# Autodesk Inventor assembly: TS_V1_Fallmagazin_gesamt
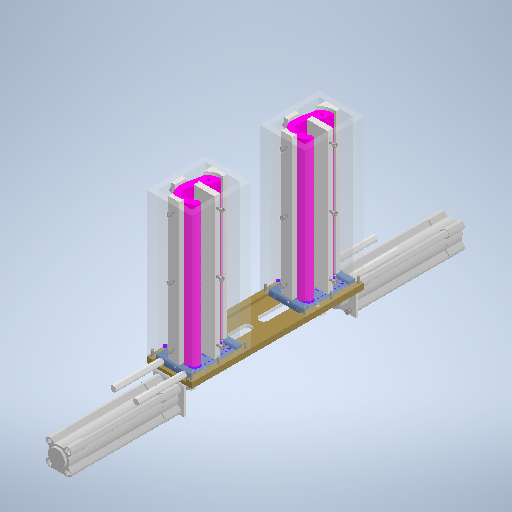
[picture p0: Inventor's stored thumbnail of the model, 512x512]
Saved by Autodesk Inventor 2025.2 (Build 292293000, 293)
## iProperties
Created: 2025-06-10
Part Number: TS_V1_Fallmagazin_gesamt
Document SubType Name: Assembly
Designer: tino
Author: tino
## Documents named in this file (16)
- C:\Users\tino\Documents_VM\Konstruieren_CAD\Useless Box\Eigene Bauteile\TS_V1_Fallmagazin_gesamt.iam
- C:\Users\tino\Documents_VM\Konstruieren_CAD\Useless Box\Eigene Bauteile\TS_V1_Fallmagazin_Boden_int.ipt
- C:\Users\tino\Documents_VM\Konstruieren_CAD\Useless Box\Eigene Bauteile\TS_V1_Fallmagazin_Wandung_int.ipt
- C:\Users\tino\Documents_VM\Konstruieren_CAD\Useless Box\Eigene Bauteile\TS_V1_Fallmagazin_Leitbleche_vorne_int.ipt
- C:\Users\tino\Documents_VM\Konstruieren_CAD\Useless Box\_Useless_Box\Finger.ipt
- C:\Users\tino\Documents_VM\Konstruieren_CAD\Useless Box\Eigene Bauteile\TS_V1_Fallmagazin_Schieber.iam
- C:\Users\tino\Documents_VM\Konstruieren_CAD\Useless Box\Kaufteile\Festo_100mm\1376426 DSBC-32-100-PPVA-N3---(0).iam
- C:\Users\tino\Documents_VM\Konstruieren_CAD\Useless Box\Kaufteile\Festo_100mm\1376426 DSBC-32-100-PPVA-N3---(0)_MIR.iam
- C:\Users\tino\Documents_VM\Konstruieren_CAD\Useless Box\Standart Bauteile\ISO 4762 - M4 x 12ISO.ipt
- C:\Users\tino\Documents_VM\Konstruieren_CAD\Useless Box\Standart Bauteile\ISO 4762 - M4 x 16ISO.ipt
- C:\Users\tino\Documents_VM\Konstruieren_CAD\Useless Box\Eigene Bauteile\TS_V1_Fallmagazin_Zylinderanbindung_int.ipt
- C:\Users\tino\Documents_VM\Konstruieren_CAD\Useless Box\Eigene Bauteile\TS_V1_Fallmagazin_Stopper_int.ipt
- C:\Users\tino\Documents_VM\Konstruieren_CAD\Useless Box\Eigene Bauteile\TS_V1_Fallmagazin_Zylinderhalter_int.ipt
- C:\Users\tino\Documents_VM\Konstruieren_CAD\Useless Box\Standart Bauteile\ISO 4762 - M5 x 8ISO.ipt
- C:\Users\tino\Documents_VM\Konstruieren_CAD\Useless Box\Standart Bauteile\ISO 4762 - M5 x 20ISO.ipt
- C:\Users\tino\Documents_VM\Konstruieren_CAD\Useless Box\Standart Bauteile\DIN EN ISO 2338 - 4 m6 x 10.ipt
## Components (169 placed, 15 different names)
1. TS_V1_Fallmagazin_Boden_int:1 — Passend:16, Passend:17, Fluchtend:5, Passend:21, Passend:23, Passend:25, Passend:26, Passend:30, Passend:31, Passend:43, Passend:44, Passend:45, Passend:46, Fluchtend:13, Passend:51, Fluchtend:15, Passend:59, Passend:60, Fluchtend:18, Passend:78, Passend:79, Passend:84, Passend:85, Passend:86, Passend:87
2. TS_V1_Fallmagazin_Wandung_int:2 — Passend:7, Passend:8, Fluchtend:4, Winkel:1, Winkel:2, Passend:16, Passend:17, Fluchtend:5, Passend:35, Passend:36, Passend:37, Passend:38, Passend:39, Passend:40, Passend:41, Passend:42, Winkel:3
3. TS_V1_Fallmagazin_Leitbleche_vorne_int:1 — Passend:7, Passend:8, Fluchtend:4, Tangential:2, Tangential:5, Fluchtend:12
4. TS_V1_Fallmagazin_Schieber:1 [sub-assembly] — Passend:21, Passend:25, Passend:26, Passend:52, Passend:53, Passend:61, Passend:62, Passend:63, Passend:64
5. TS_V1_Fallmagazin_Schieber:2 [sub-assembly] — Passend:23, Passend:30, Passend:31, Passend:56, Passend:57, Passend:65, Passend:66, Passend:67
6. 1376426 DSBC-32-100-PPVA-N3---(0):1 [sub-assembly] — Passend:54, Passend:59, Fluchtend:17, Fluchtend:18, Passend:68, Passend:69, Passend:70
7. 1376426 DSBC-32-100-PPVA-N3---(0)_MIR:1 [sub-assembly] — Passend:51, Fluchtend:15, Passend:58, Passend:60, Fluchtend:17, Passend:75, Passend:76, Passend:77
8. TS_V1_Fallmagazin_Wandung_int:3 — Passend:45, Passend:46, Fluchtend:13, Passend:47, Fluchtend:14, Passend:48
9. TS_V1_Fallmagazin_Leitbleche_vorne_int:2 — Passend:47, Fluchtend:14, Passend:48
10. TS_V1_Fallmagazin_Zylinderanbindung_int:1 — Passend:52, Passend:53, Passend:54
11. TS_V1_Fallmagazin_Zylinderanbindung_int:2 — Passend:56, Passend:57, Passend:58
12. TS_V1_Fallmagazin_Stopper_int:1 — Passend:61, Passend:62, Winkel:3
13. TS_V1_Fallmagazin_Stopper_int:2 — Passend:63, Passend:64
14. TS_V1_Fallmagazin_Stopper_int:3 — Passend:65, Fluchtend:16, Passend:67
15. TS_V1_Fallmagazin_Stopper_int:4 — Passend:66, Fluchtend:16
16. TS_V1_Fallmagazin_Zylinderhalter_int:1 — Passend:68, Passend:69, Passend:70, Passend:71, Passend:72, Passend:73, Passend:74
17. TS_V1_Fallmagazin_Zylinderhalter_int:2 — Passend:75, Passend:76, Passend:77, Passend:78, Passend:79, Passend:80, Passend:81, Passend:82, Passend:83
18. DIN EN ISO 2338 4 m6 x 10:1 — Passend:84, Passend:85
19. DIN EN ISO 2338 4 m6 x 10:2 — Passend:86, Passend:87
20. Finger:1 — Winkel:1, Tangential:2, Tangential:5, Winkel:2, Fluchtend:12
21. Finger:2
22. Finger:3
23. Finger:4
24. Finger:5
25. Finger:6
26. Finger:7
27. Finger:8
28. Finger:9
29. Finger:10
30. Finger:11
31. Finger:12
32. Finger:13
33. Finger:14
34. Finger:15
35. Finger:16
36. Finger:17
37. Finger:18
38. Finger:19
39. Finger:20
40. Finger:21
41. Finger:22
42. Finger:23
43. Finger:24
44. Finger:25
45. Finger:26
46. Finger:27
47. Finger:28
48. Finger:29
49. Finger:30
50. Finger:31
51. Finger:32
52. Finger:33
53. Finger:34
54. Finger:35
55. Finger:36
56. Finger:37
57. Finger:38
58. Finger:39
59. Finger:40
60. Finger:41
61. Finger:42
62. Finger:43
63. Finger:44
64. Finger:45
65. Finger:46
66. Finger:47
67. Finger:48
68. Finger:49
69. Finger:50
70. Finger:51
71. Finger:52
72. Finger:53
73. Finger:54
74. Finger:55
75. Finger:56
76. Finger:57
77. Finger:58
78. Finger:59
79. Finger:60
80. Finger:61
81. Finger:62
82. Finger:63
83. Finger:64
84. Finger:65
85. Finger:66
86. Finger:67
87. Finger:68
88. Finger:69
89. Finger:70
90. Finger:71
91. Finger:72
92. Finger:73
93. Finger:74
94. Finger:75
95. Finger:76
96. Finger:77
97. Finger:78
98. Finger:79
99. Finger:80
100. Finger:81
101. Finger:82
102. Finger:83
103. Finger:84
104. Finger:85
105. Finger:86
106. Finger:87
107. Finger:88
108. Finger:89
109. Finger:90
110. Finger:91
111. Finger:92
112. Finger:93
113. Finger:94
114. Finger:95
115. Finger:96
116. Finger:97
117. Finger:98
118. ISO 4762 M5 x 8:1 — Passend:71, Passend:72
119. ISO 4762 M5 x 8:2
120. ISO 4762 M5 x 8:3
121. ISO 4762 M5 x 8:4
122. ISO 4762 M5 x 20:1 — Passend:73, Passend:74
123. ISO 4762 M5 x 20:2
124. ISO 4762 M5 x 20:3
125. ISO 4762 M5 x 20:4
126. ISO 4762 M5 x 8:5 — Passend:80, Passend:81
127. ISO 4762 M5 x 8:6
128. ISO 4762 M5 x 8:7
129. ISO 4762 M5 x 8:8
130. ISO 4762 M5 x 20:5 — Passend:82, Passend:83
131. ISO 4762 M5 x 20:6
132. ISO 4762 M5 x 20:7
133. ISO 4762 M5 x 20:8
134. ISO 4762 M4 x 12:1 — Passend:35, Passend:36
135. ISO 4762 M4 x 12:2
136. ISO 4762 M4 x 12:3
137. ISO 4762 M4 x 12:4 — Passend:37, Passend:38
138. ISO 4762 M4 x 12:5
139. ISO 4762 M4 x 12:6
140. ISO 4762 M4 x 12:7 — Passend:39, Passend:40
141. ISO 4762 M4 x 12:8
142. ISO 4762 M4 x 12:9
143. ISO 4762 M4 x 12:10 — Passend:41, Passend:42
144. ISO 4762 M4 x 12:11
145. ISO 4762 M4 x 12:12
146. ISO 4762 M4 x 16:1 — Passend:43, Passend:44
147. ISO 4762 M4 x 16:2
148. ISO 4762 M4 x 16:3
149. ISO 4762 M4 x 16:4
150. ISO 4762 M4 x 16:5
151. ISO 4762 M4 x 16:6
152. ISO 4762 M4 x 12:13
153. ISO 4762 M4 x 12:14
154. ISO 4762 M4 x 12:15
155. ISO 4762 M4 x 12:16
156. ISO 4762 M4 x 12:17
157. ISO 4762 M4 x 12:18
158. ISO 4762 M4 x 12:19
159. ISO 4762 M4 x 12:20
160. ISO 4762 M4 x 12:21
161. ISO 4762 M4 x 12:22
162. ISO 4762 M4 x 12:23
163. ISO 4762 M4 x 12:24
164. ISO 4762 M4 x 16:7
165. ISO 4762 M4 x 16:8
166. ISO 4762 M4 x 16:9
167. ISO 4762 M4 x 16:10
168. ISO 4762 M4 x 16:11
169. ISO 4762 M4 x 16:12
## Component patterns: (2 elements), (98 elements, first: Finger:1), (4 elements, first: ISO 4762 M5 x 8:1), (4 elements, first: ISO 4762 M5 x 20:1), (4 elements, first: ISO 4762 M5 x 8:5), (4 elements, first: ISO 4762 M5 x 20:5), (3 elements, first: ISO 4762 M4 x 12:1), (3 elements, first: ISO 4762 M4 x 12:4), (3 elements, first: ISO 4762 M4 x 12:7), (3 elements, first: ISO 4762 M4 x 12:10), (6 elements, first: ISO 4762 M4 x 16:1), Komponentenanordnung 2:2 (3 elements), Komponentenanordnung 3:2 (3 elements), Komponentenanordnung 4:2 (3 elements), Komponentenanordnung 5:2 (3 elements), Komponentenanordnung 6:2 (6 elements)
## Relationships (74: Mate 60, Flush 9, Angle 3, Tangent 2)
- Passend:7 [Mate]: TS_V1_Fallmagazin_Wandung_int:2 ↔ TS_V1_Fallmagazin_Leitbleche_vorne_int:1
- Passend:8 [Mate]: TS_V1_Fallmagazin_Wandung_int:2 ↔ TS_V1_Fallmagazin_Leitbleche_vorne_int:1
- Fluchtend:4 [Flush]: TS_V1_Fallmagazin_Wandung_int:2 ↔ TS_V1_Fallmagazin_Leitbleche_vorne_int:1
- Winkel:1 [Angle] (0 deg): TS_V1_Fallmagazin_Wandung_int:2 ↔ Finger:1
- Tangential:2: TS_V1_Fallmagazin_Leitbleche_vorne_int:1 ↔ Finger:1
- Tangential:5: TS_V1_Fallmagazin_Leitbleche_vorne_int:1 ↔ Finger:1
- Winkel:2 [Angle] (0 deg): TS_V1_Fallmagazin_Wandung_int:2 ↔ Finger:1
- Passend:16 [Mate]: TS_V1_Fallmagazin_Boden_int:1 ↔ TS_V1_Fallmagazin_Wandung_int:2
- Passend:17 [Mate]: TS_V1_Fallmagazin_Boden_int:1 ↔ TS_V1_Fallmagazin_Wandung_int:2
- Fluchtend:5 [Flush]: TS_V1_Fallmagazin_Boden_int:1 ↔ TS_V1_Fallmagazin_Wandung_int:2
- Passend:21 [Mate]: TS_V1_Fallmagazin_Boden_int:1 ↔ TS_V1_Fallmagazin_Schieber:1
- Passend:23 [Mate]: TS_V1_Fallmagazin_Boden_int:1 ↔ TS_V1_Fallmagazin_Schieber:2
- Passend:25 [Mate]: TS_V1_Fallmagazin_Boden_int:1 ↔ TS_V1_Fallmagazin_Schieber:1
- Passend:26 [Mate]: TS_V1_Fallmagazin_Boden_int:1 ↔ TS_V1_Fallmagazin_Schieber:1
- Passend:30 [Mate]: TS_V1_Fallmagazin_Boden_int:1 ↔ TS_V1_Fallmagazin_Schieber:2
- Passend:31 [Mate]: TS_V1_Fallmagazin_Boden_int:1 ↔ TS_V1_Fallmagazin_Schieber:2
- Passend:35 [Mate]: TS_V1_Fallmagazin_Wandung_int:2 ↔ ISO 4762 M4 x 12:1
- Passend:36 [Mate]: TS_V1_Fallmagazin_Wandung_int:2 ↔ ISO 4762 M4 x 12:1
- Passend:37 [Mate]: TS_V1_Fallmagazin_Wandung_int:2 ↔ ISO 4762 M4 x 12:4
- Passend:38 [Mate]: TS_V1_Fallmagazin_Wandung_int:2 ↔ ISO 4762 M4 x 12:4
- Passend:39 [Mate]: TS_V1_Fallmagazin_Wandung_int:2 ↔ ISO 4762 M4 x 12:7
- Passend:40 [Mate]: TS_V1_Fallmagazin_Wandung_int:2 ↔ ISO 4762 M4 x 12:7
- Passend:41 [Mate]: TS_V1_Fallmagazin_Wandung_int:2 ↔ ISO 4762 M4 x 12:10
- Passend:42 [Mate]: TS_V1_Fallmagazin_Wandung_int:2 ↔ ISO 4762 M4 x 12:10
- Passend:43 [Mate]: TS_V1_Fallmagazin_Boden_int:1 ↔ ISO 4762 M4 x 16:1
- Passend:44 [Mate]: TS_V1_Fallmagazin_Boden_int:1 ↔ ISO 4762 M4 x 16:1
- Fluchtend:12 [Flush]: TS_V1_Fallmagazin_Leitbleche_vorne_int:1 ↔ Finger:1
- Passend:45 [Mate]: TS_V1_Fallmagazin_Boden_int:1 ↔ TS_V1_Fallmagazin_Wandung_int:3
- Passend:46 [Mate]: TS_V1_Fallmagazin_Boden_int:1 ↔ TS_V1_Fallmagazin_Wandung_int:3
- Fluchtend:13 [Flush]: TS_V1_Fallmagazin_Boden_int:1 ↔ TS_V1_Fallmagazin_Wandung_int:3
- Passend:47 [Mate]: TS_V1_Fallmagazin_Wandung_int:3 ↔ TS_V1_Fallmagazin_Leitbleche_vorne_int:2
- Fluchtend:14 [Flush]: TS_V1_Fallmagazin_Wandung_int:3 ↔ TS_V1_Fallmagazin_Leitbleche_vorne_int:2
- Passend:48 [Mate]: TS_V1_Fallmagazin_Wandung_int:3 ↔ TS_V1_Fallmagazin_Leitbleche_vorne_int:2
- Passend:51 [Mate] (4 mm): TS_V1_Fallmagazin_Boden_int:1 ↔ 1376426 DSBC-32-100-PPVA-N3---(0)_MIR:1
- Fluchtend:15 [Flush]: TS_V1_Fallmagazin_Boden_int:1 ↔ 1376426 DSBC-32-100-PPVA-N3---(0)_MIR:1
- Passend:52 [Mate]: TS_V1_Fallmagazin_Schieber:1 ↔ TS_V1_Fallmagazin_Zylinderanbindung_int:1
- Passend:53 [Mate]: TS_V1_Fallmagazin_Schieber:1 ↔ TS_V1_Fallmagazin_Zylinderanbindung_int:1
- Passend:54 [Mate]: 1376426 DSBC-32-100-PPVA-N3---(0):1 ↔ TS_V1_Fallmagazin_Zylinderanbindung_int:1
- Passend:56 [Mate]: TS_V1_Fallmagazin_Schieber:2 ↔ TS_V1_Fallmagazin_Zylinderanbindung_int:2
- Passend:57 [Mate]: TS_V1_Fallmagazin_Schieber:2 ↔ TS_V1_Fallmagazin_Zylinderanbindung_int:2
- Passend:58 [Mate]: 1376426 DSBC-32-100-PPVA-N3---(0)_MIR:1 ↔ TS_V1_Fallmagazin_Zylinderanbindung_int:2
- Passend:59 [Mate] (-16.4 mm): TS_V1_Fallmagazin_Boden_int:1 ↔ 1376426 DSBC-32-100-PPVA-N3---(0):1
- Passend:60 [Mate] (-16.4 mm): TS_V1_Fallmagazin_Boden_int:1 ↔ 1376426 DSBC-32-100-PPVA-N3---(0)_MIR:1
- Passend:61 [Mate]: TS_V1_Fallmagazin_Schieber:1 ↔ TS_V1_Fallmagazin_Stopper_int:1
- Passend:62 [Mate]: TS_V1_Fallmagazin_Schieber:1 ↔ TS_V1_Fallmagazin_Stopper_int:1
- Passend:63 [Mate]: TS_V1_Fallmagazin_Schieber:1 ↔ TS_V1_Fallmagazin_Stopper_int:2
- Passend:64 [Mate]: TS_V1_Fallmagazin_Schieber:1 ↔ TS_V1_Fallmagazin_Stopper_int:2
- Passend:65 [Mate]: TS_V1_Fallmagazin_Schieber:2 ↔ TS_V1_Fallmagazin_Stopper_int:3
- Passend:66 [Mate]: TS_V1_Fallmagazin_Schieber:2 ↔ TS_V1_Fallmagazin_Stopper_int:4
- Fluchtend:16 [Flush]: TS_V1_Fallmagazin_Stopper_int:3 ↔ TS_V1_Fallmagazin_Stopper_int:4
- Passend:67 [Mate]: TS_V1_Fallmagazin_Schieber:2 ↔ TS_V1_Fallmagazin_Stopper_int:3
- Fluchtend:17 [Flush]: 1376426 DSBC-32-100-PPVA-N3---(0):1 ↔ 1376426 DSBC-32-100-PPVA-N3---(0)_MIR:1
- Fluchtend:18 [Flush]: TS_V1_Fallmagazin_Boden_int:1 ↔ 1376426 DSBC-32-100-PPVA-N3---(0):1
- Passend:68 [Mate]: 1376426 DSBC-32-100-PPVA-N3---(0):1 ↔ TS_V1_Fallmagazin_Zylinderhalter_int:1
- Passend:69 [Mate]: 1376426 DSBC-32-100-PPVA-N3---(0):1 ↔ TS_V1_Fallmagazin_Zylinderhalter_int:1
- Passend:70 [Mate]: 1376426 DSBC-32-100-PPVA-N3---(0):1 ↔ TS_V1_Fallmagazin_Zylinderhalter_int:1
- Passend:71 [Mate]: TS_V1_Fallmagazin_Zylinderhalter_int:1 ↔ ISO 4762 M5 x 8:1
- Passend:72 [Mate]: TS_V1_Fallmagazin_Zylinderhalter_int:1 ↔ ISO 4762 M5 x 8:1
- Passend:73 [Mate]: TS_V1_Fallmagazin_Zylinderhalter_int:1 ↔ ISO 4762 M5 x 20:1
- Passend:74 [Mate]: TS_V1_Fallmagazin_Zylinderhalter_int:1 ↔ ISO 4762 M5 x 20:1
- Passend:75 [Mate]: 1376426 DSBC-32-100-PPVA-N3---(0)_MIR:1 ↔ TS_V1_Fallmagazin_Zylinderhalter_int:2
- Passend:76 [Mate]: 1376426 DSBC-32-100-PPVA-N3---(0)_MIR:1 ↔ TS_V1_Fallmagazin_Zylinderhalter_int:2
- Passend:77 [Mate]: 1376426 DSBC-32-100-PPVA-N3---(0)_MIR:1 ↔ TS_V1_Fallmagazin_Zylinderhalter_int:2
- Passend:78 [Mate]: TS_V1_Fallmagazin_Boden_int:1 ↔ TS_V1_Fallmagazin_Zylinderhalter_int:2
- Passend:79 [Mate]: TS_V1_Fallmagazin_Boden_int:1 ↔ TS_V1_Fallmagazin_Zylinderhalter_int:2
- Passend:80 [Mate]: TS_V1_Fallmagazin_Zylinderhalter_int:2 ↔ ISO 4762 M5 x 8:5
- Passend:81 [Mate]: TS_V1_Fallmagazin_Zylinderhalter_int:2 ↔ ISO 4762 M5 x 8:5
- Passend:82 [Mate]: TS_V1_Fallmagazin_Zylinderhalter_int:2 ↔ ISO 4762 M5 x 20:5
- Passend:83 [Mate]: TS_V1_Fallmagazin_Zylinderhalter_int:2 ↔ ISO 4762 M5 x 20:5
- Passend:84 [Mate]: TS_V1_Fallmagazin_Boden_int:1 ↔ DIN EN ISO 2338 4 m6 x 10:1
- Passend:85 [Mate] (0.5 mm): TS_V1_Fallmagazin_Boden_int:1 ↔ DIN EN ISO 2338 4 m6 x 10:1
- Passend:86 [Mate]: TS_V1_Fallmagazin_Boden_int:1 ↔ DIN EN ISO 2338 4 m6 x 10:2
- Passend:87 [Mate] (1 mm): TS_V1_Fallmagazin_Boden_int:1 ↔ DIN EN ISO 2338 4 m6 x 10:2
- Winkel:3 [Angle] (0 deg): TS_V1_Fallmagazin_Wandung_int:2 ↔ TS_V1_Fallmagazin_Stopper_int:1
## Named parameters: Magazin_Hoehe = 255 mm, Abstand_Schrauben_vert = 105 mm, Abstand_Rand = 45 mm, Anbindung_Zylinder = 16.4 mm
